# Autodesk Inventor assembly: 2024-210-Angle-Shootaur
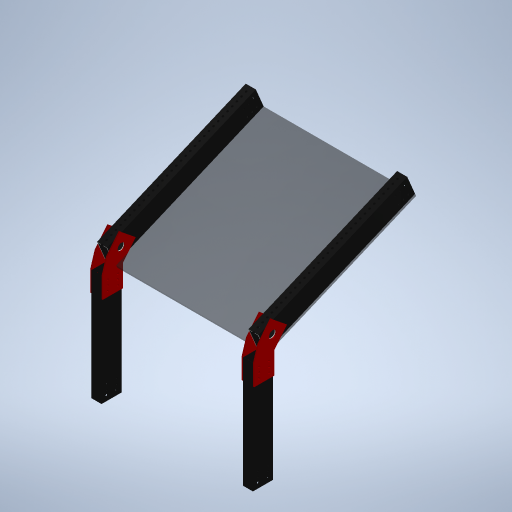
[picture p0: Inventor's stored thumbnail of the model, 512x512]
Saved by Autodesk Inventor 2024 (Build 280153000, 153)
## iProperties
Created: 2024-01-23
Part Number: 2024-210-Angle-Shootaur
Document SubType Name: Assembly
Designer: rohan
Author: rohan
## Documents named in this file (5)
- C:\Users\5652160\OneDrive - Hillsborough County Public Schools\Robotics\FIRST-Robotics-Competition\Crescendo\Minotaur-Crescendo-Robot\Structure\Superstructure\Angle-Shootaur\2024-210-Angle-Shootaur.iam
- C:\Users\5652160\OneDrive - Hillsborough County Public Schools\Robotics\FIRST-Robotics-Competition\Crescendo\Minotaur-Crescendo-Robot\Structure\Superstructure\Angle-Shootaur\2024-210-003-Dead-Axle-Gusset_1.ipt
- C:\Users\5652160\OneDrive - Hillsborough County Public Schools\Robotics\FIRST-Robotics-Competition\Crescendo\Minotaur-Crescendo-Robot\Structure\Superstructure\Angle-Shootaur\2024-210-002-Angle-Beam_1.ipt
- C:\Users\5652160\OneDrive - Hillsborough County Public Schools\Robotics\FIRST-Robotics-Competition\Crescendo\Minotaur-Crescendo-Robot\Structure\Superstructure\Angle-Shootaur\2024-210-001-Backright-Support_1.ipt
- C:\Users\5652160\OneDrive - Hillsborough County Public Schools\Robotics\FIRST-Robotics-Competition\Crescendo\Minotaur-Crescendo-Robot\Structure\Superstructure\Polycarbonate-Note-Rest.ipt
## Components (9 placed, 4 different names)
1. 2024-210-002-Angle-Beam_1:1 — Flush:8, Mate:7, Mate:9, Flush:12, Mate:10, Mate:11
2. 2024-210-003-Dead-Axle-Gusset_1:3 — Flush:1, Flush:2, Mate:1, Insert:1, Insert:2
3. 2024-210-003-Dead-Axle-Gusset_1:4 — Flush:1, Flush:2, Mate:1, Mate:3
4. 2024-210-002-Angle-Beam_1:2 — Mate:6, Flush:6, Flush:11
5. 2024-210-001-Backright-Support_1:2 — Mate:3, Insert:1, Insert:2, Flush:9, Flush:10, Mate:8
6. Polycarbonate-Note-Rest:1 — Mate:6, Flush:6, Flush:8, Mate:7, Flush:11, Flush:12
7. 2024-210-003-Dead-Axle-Gusset_1:5 — Mate:9, Mate:10, Mate:11
8. 2024-210-003-Dead-Axle-Gusset_1:6
9. 2024-210-001-Backright-Support_1:3 — Flush:9, Flush:10, Mate:8
## Relationships (24: Flush 10, Mate 10, Insert 4)
- Flush:1: 2024-210-003-Dead-Axle-Gusset_1:3 ↔ 2024-210-003-Dead-Axle-Gusset_1:4
- Flush:2: 2024-210-003-Dead-Axle-Gusset_1:3 ↔ 2024-210-003-Dead-Axle-Gusset_1:4
- Mate:1 (25.4 mm): 2024-210-003-Dead-Axle-Gusset_1:3 ↔ 2024-210-003-Dead-Axle-Gusset_1:4
- Mate:3: 2024-210-003-Dead-Axle-Gusset_1:4 ↔ 2024-210-001-Backright-Support_1:2
- Insert:1: 2024-210-003-Dead-Axle-Gusset_1:3 ↔ 2024-210-001-Backright-Support_1:2
- Insert:2: 2024-210-003-Dead-Axle-Gusset_1:3 ↔ 2024-210-001-Backright-Support_1:2
- [Flush]: 2024-210-003-Dead-Axle-Gusset_1:5 ↔ 2024-210-003-Dead-Axle-Gusset_1:6
- [Flush]: 2024-210-003-Dead-Axle-Gusset_1:5 ↔ 2024-210-003-Dead-Axle-Gusset_1:6
- [Mate] (25.4 mm): 2024-210-003-Dead-Axle-Gusset_1:5 ↔ 2024-210-003-Dead-Axle-Gusset_1:6
- [Mate]: 2024-210-003-Dead-Axle-Gusset_1:6 ↔ 2024-210-001-Backright-Support_1:3
- [Insert]: 2024-210-003-Dead-Axle-Gusset_1:5 ↔ 2024-210-001-Backright-Support_1:3
- [Insert]: 2024-210-003-Dead-Axle-Gusset_1:5 ↔ 2024-210-001-Backright-Support_1:3
- Mate:6: 2024-210-002-Angle-Beam_1:2 ↔ Polycarbonate-Note-Rest:1
- Flush:6: 2024-210-002-Angle-Beam_1:2 ↔ Polycarbonate-Note-Rest:1
- Flush:8: 2024-210-002-Angle-Beam_1:1 ↔ Polycarbonate-Note-Rest:1
- Mate:7: 2024-210-002-Angle-Beam_1:1 ↔ Polycarbonate-Note-Rest:1
- Flush:9: 2024-210-001-Backright-Support_1:2 ↔ 2024-210-001-Backright-Support_1:3
- Flush:10: 2024-210-001-Backright-Support_1:2 ↔ 2024-210-001-Backright-Support_1:3
- Mate:8 (355.6 mm): 2024-210-001-Backright-Support_1:2 ↔ 2024-210-001-Backright-Support_1:3
- Mate:9: 2024-210-002-Angle-Beam_1:1 ↔ 2024-210-003-Dead-Axle-Gusset_1:5
- Flush:11: 2024-210-002-Angle-Beam_1:2 ↔ Polycarbonate-Note-Rest:1
- Flush:12: 2024-210-002-Angle-Beam_1:1 ↔ Polycarbonate-Note-Rest:1
- Mate:10: 2024-210-002-Angle-Beam_1:1 ↔ 2024-210-003-Dead-Axle-Gusset_1:5
- Mate:11: 2024-210-002-Angle-Beam_1:1 ↔ 2024-210-003-Dead-Axle-Gusset_1:5
## Named parameters: d43_d40 = 0 mm, d44_d41 = 0 mm, d45_d42 = 0 mm, d46_d34 = 0 mm, d47_d35 = 0 mm, d48_d36 = 25.4 mm
